# Autodesk Inventor assembly: SCHUNK- 1321170 Co-act EGP-C 40-N-N-KTOE, 0
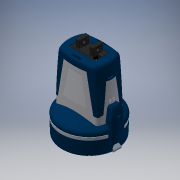
[picture p0: Inventor's stored thumbnail of the model, 180x180]
Saved by Autodesk Inventor 2019 (Build 230136000, 136)
## iProperties
Category: PARTsolutions
Company: SCHUNK
Created: 2022-08-29
Part Number: SCHUNK- 1321170 Co-act EGP-C 40-N-N-KTOE, 0
Catalog Web Link: www.cadenas.de
Description: Co-act EGP-C-Collaborating gripper for small components
Vendor: SCHUNK
Document SubType Name: Assembly
Designer: psAdmin
Manufacturer: SCHUNK
Mass: 620 g
Surface Area: 1018.14 cm^2
Volume: 436.323 cm^3
Density: 1.42097 g/cm^3
Title: SCHUNK-1321170 Co-act EGP-C 40-N-N-KTOE
Author: Cadenas PARTsolutions
Comments: Collaborating gripper for small components
PSOL_IDENT_0: {$CADENAS_DATA/23d-libs/schunk/greifsysteme/greifmodule/co_act/co_act_egp_c/co_act_egp_c_asm_at.prj}
PSOL_IDENT_1: ,248 {VTYP=3D},{STYP=ASSTAB},{NB=SCHUNK- 1321170 Co-act EGP-C 40-N-N-KTOE, 0},{LINA=SCHUNK-1321170 C
PSOL_IDENT_2: o-act EGP-C 40-N-N-KTOE},{NN=Co-act EGP-C},{DATE=01.06.2022 15:24:31},{GEOMDATE=27.04.2022 08:42:34}
PSOL_IDENT_3: ,{VERSION=},{LINEID=20},{WBVAR=HUB},{WBNUMERIC=HUB}  {NB=SCHUNK- 1321170 Co-act EGP-C 40-N-N-KTOE, 0
PSOL_IDENT_4: },{LINA=SCHUNK-1321170 Co-act EGP-C 40-N-N-KTOE},{KT=DUMMY},{IDNR=1321170},{TYP=Co-act EGP-C 40-N-N-
PSOL_IDENT_5: KTOE},{ONLINE=Zur Produktseite},{INFOXX=https://schunk.com/gb_en/gripping-systems/product/63294-0},{
PSOL_IDENT_6: HUB=0},{CALC=../../../../produktbilder/icons/im0023672.png},{EPLAN=../../../../produktbilder/icons/i
PSOL_IDENT_7: m0021678.png},{HUBMAX=6.000},{PARTSERVER=1.000},{TYPBG=2.000},{TYP1=1.000},{TYPFLA=2.000},{WFLA=30.0
PSOL_IDENT_8: 00},{TYPEGP=EGP 40-N-N-B},{ROBOTER=KUKA LBR iiwa 7/14},{FLANSCH=Medien-Flansch Touch elektrisch},{LE
PSOL_IDENT_9: D=integriert},{FARBEN=Grün, Gelb, Rot},{SENSOREN=Ja, 2-fach induktiv},{HUBBACKE=6},{GREIFKRAFT=35/14
PSOL_IDENT_10: 0},{KRAFTPROBACKE=17.5/70},{WKSTGEWICHT=0.700},{FINGERLAENGE=50},{MASSEFINGER=0.080},{WIEDERHOLGENAU
PSOL_IDENT_11: I=0.020},{SCHLIESSOEFFNUN=0.2/0.2},{EIGENMASSE=0.620},{UMGEBUNGSTEMPER=5/55},{SCHUTZART=30},{KABELST
PSOL_IDENT_12: ECKEREND=M12},{KABELLAENGE=70},{NENNSPANN=24},{NENNSTROM=0.200},{MAXSTROM=2.000},{REGLERELEKTRONI=in
PSOL_IDENT_13: tegriert},{KOMMUNIKATIONSS=Digitale I/O},{ANZDIGITALEIO=4/2},{HOEHE=118.000},{HEGP=88.500},{CALCXX=h
PSOL_IDENT_14: ttps://schunk.com/de_de/services/digitale-services/berechnungs-und-auslegungstool-greifen/},{CALCXXX=
PSOL_IDENT_15: https://schunk.com/de_de/services/digitale-services/berechnungs-und-auslegungstool-greifen/},{EPLANX
PSOL_IDENT_16: X=https://eplandata.de/portal/portal.php?action=part-viewc&edpp=1.0&ev=1.9.11&lang=de_DE&clang=de_DE
PSOL_IDENT_17: &mf=SNK&lastmpg=.&mcat=_eplan&tab=c&mcatsel=SNK},{EPLANXXX=https://eplandata.de/portal/portal.php?ac
PSOL_IDENT_18: tion=part-viewc&edpp=1.0&ev=1.9.11&lang=de_DE&clang=de_DE&mf=SNK&lastmpg=.&mcat=_eplan&tab=c&mcatsel=
PSOL_IDENT_19: SNK},{CNSCTN=84798997},{EDZ=snk.1321170},{EPIMID=63294},{PPATH=co_act_egp_c_asmsbl.prj}
NB: SCHUNK- 1321170 Co-act EGP-C 40-N-N-KTOE, 0
NN: Co-act EGP-C
NT: Collaborating gripper for small components
NBSYN: SCHUNK- $IDNR. $TYP., $HUB.
LINA: SCHUNK-1321170 Co-act EGP-C 40-N-N-KTOE
CATALOG: SCHUNK
IDNR: 1321170
TYP: Co-act EGP-C 40-N-N-KTOE
ONLINE: To the product page
HUB: 0
CALC: ../../../../produktbilder/icons/im0023672.png
EPLAN: ../../../../produktbilder/icons/im0021678.png
ROBOTER: KUKA LBR iiwa 7/14
FLANSCH: Media flange touch electric
LED: integrated
FARBEN: green, yellow, red
SENSOREN: yes, inductive in two directions
HUBBACKE: 6
GREIFKRAFT: 35/140
KRAFTPROBACKE: 17.5/70
WKSTGEWICHT: 0.7
FINGERLAENGE: 50
MASSEFINGER: 0.08
WIEDERHOLGENAUI: 0.02
SCHLIESSOEFFNUN: 0.2/0.2
EIGENMASSE: 0.62
UMGEBUNGSTEMPER: 5/55
SCHUTZART: 30
KABELSTECKEREND: M12
KABELLAENGE: 70
NENNSPANN: 24
NENNSTROM: 0.2
MAXSTROM: 2
REGLERELEKTRONI: integrated
KOMMUNIKATIONSS: digital I/O
ANZDIGITALEIO: 4/2
CNSCTN: 84798997
SUPPLIER: SCHUNK
ARTICLENO: SCHUNK- 1321170 Co-act EGP-C 40-N-N-KTOE, 0
BOMINFO: SCHUNK-1321170 Co-act EGP-C 40-N-N-KTOE
CREATOR: CADENAS GmbH
## Documents named in this file (11)
- e:\temp\worker_COMMON_2\temp\exporttempdir_6540_146_MRx3B\format_0\SCHUNK- 1321170 Co-act EGP-C 40-N-N-KTOE, 0.iam
- e:\temp\worker_COMMON_2\temp\exporttempdir_6540_146_MRx3B\format_0\Co-act EGP-C 40 Modell 1.ipt
- e:\temp\worker_COMMON_2\temp\exporttempdir_6540_146_MRx3B\format_0\SCHUNK-1013180-ISO-1-50-M6 Universalflansch Co-act-EGP-C.ipt
- e:\temp\worker_COMMON_2\temp\exporttempdir_6540_146_MRx3B\format_0\SCHUNK-9905502 Typenschild 9x24x0_3.ipt
- e:\temp\worker_COMMON_2\temp\exporttempdir_6540_146_MRx3B\format_0\SCHUNK-5521120 Gehaeuse EGP 40.ipt
- e:\temp\worker_COMMON_2\temp\exporttempdir_6540_146_MRx3B\format_0\SCHUNK-SNT016581 Stecker EGP.ipt
- e:\temp\worker_COMMON_2\temp\exporttempdir_6540_146_MRx3B\format_0\SCHUNK-9700901 Halter fuer NHS Du 4.ipt
- e:\temp\worker_COMMON_2\temp\exporttempdir_6540_146_MRx3B\format_0\SCHUNK-5521119 Finger EGP 40.ipt
- e:\temp\worker_COMMON_2\temp\exporttempdir_6540_146_MRx3B\format_0\SCHUNK-9962713 Bracket MPG 40.ipt
- e:\temp\worker_COMMON_2\temp\exporttempdir_6540_146_MRx3B\format_0\SCHUNK-9965221-Scheibe D4_5.ipt
- e:\temp\worker_COMMON_2\temp\exporttempdir_6540_146_MRx3B\format_0\SCHUNK-5509536 Huelse MPG 40.ipt
## Components (18 placed, 10 different names)
1. Co-act EGP-C 40 Modell 1:1 — fla_XY@1 <-> fla_XY@2, fla_Z@1 <-> fla_Z@2, fla_YZ@1 <-> fla_YZ@2, typ_XY@1 <-> aluschild_XY@3, typ_Z@1 <-> aluschild_Z@3, typ_YZ@1 <-> aluschild_YZ@3
2. SCHUNK-1013180-ISO-1-50-M6 Universalflansch Co-act-EGP-C:1 — fla_XY@1 <-> fla_XY@2, fla_Z@1 <-> fla_Z@2, fla_YZ@1 <-> fla_YZ@2
3. SCHUNK-9905502 Typenschild 9x24x0_3:1 — typ_XY@1 <-> aluschild_XY@3, typ_Z@1 <-> aluschild_Z@3, typ_YZ@1 <-> aluschild_YZ@3
4. SCHUNK-5521120 Gehaeuse EGP 40:1 — hal_nhs_1_XY@4 <-> as_nhs_02_XY@6, hal_nhs_1_Z@4 <-> as_nhs_02_Z@6, hal_nhs_1_YZ@4 <-> as_nhs_02_YZ@6, fin_1_XY@4 <-> HUB_XY@8, fin_1_Z@4 <-> HUB_Z@8, fin_1_YZ@4 <-> HUB_YZ@8, fin_2_XY@4 <-> HUB_XY@13, fin_2_Z@4 <-> HUB_Z@13, fin_2_YZ@4 <-> HUB_YZ@13, typ_XY@4 <-> aluschild_XY@18, typ_Z@4 <-> aluschild_Z@18, typ_YZ@4 <-> aluschild_YZ@18
5. SCHUNK-SNT016581 Stecker EGP:1
6. SCHUNK-9700901 Halter fuer NHS Du 4:1 — hal_nhs_1_XY@4 <-> as_nhs_02_XY@6, hal_nhs_1_Z@4 <-> as_nhs_02_Z@6, hal_nhs_1_YZ@4 <-> as_nhs_02_YZ@6
7. SCHUNK-9700901 Halter fuer NHS Du 4:2
8. SCHUNK-5521119 Finger EGP 40:1 — fin_1_XY@4 <-> HUB_XY@8, fin_1_Z@4 <-> HUB_Z@8, fin_1_YZ@4 <-> HUB_YZ@8, hal_1_XY@8 <-> hal_XY@9, hal_1_Z@8 <-> hal_Z@9, hal_1_YZ@8 <-> hal_YZ@9, hal_2_XY@8 <-> hal_XY@11, hal_2_Z@8 <-> hal_Z@11, hal_2_YZ@8 <-> hal_YZ@11
9. SCHUNK-9962713 Bracket MPG 40:1 — hal_1_XY@8 <-> hal_XY@9, hal_1_Z@8 <-> hal_Z@9, hal_1_YZ@8 <-> hal_YZ@9, s01_XY@9 <-> hal_XY@10, s01_Z@9 <-> hal_Z@10, s01_YZ@9 <-> hal_YZ@10
10. SCHUNK-9965221-Scheibe D4_5:1 — s01_XY@9 <-> hal_XY@10, s01_Z@9 <-> hal_Z@10, s01_YZ@9 <-> hal_YZ@10
11. SCHUNK-9962713 Bracket MPG 40:2 — hal_2_XY@8 <-> hal_XY@11, hal_2_Z@8 <-> hal_Z@11, hal_2_YZ@8 <-> hal_YZ@11, s01_XY@11 <-> hal_XY@12, s01_Z@11 <-> hal_Z@12, s01_YZ@11 <-> hal_YZ@12
12. SCHUNK-9965221-Scheibe D4_5:2 — s01_XY@11 <-> hal_XY@12, s01_Z@11 <-> hal_Z@12, s01_YZ@11 <-> hal_YZ@12
13. SCHUNK-5521119 Finger EGP 40:2 — fin_2_XY@4 <-> HUB_XY@13, fin_2_Z@4 <-> HUB_Z@13, fin_2_YZ@4 <-> HUB_YZ@13, hal_1_XY@13 <-> hal_XY@14, hal_1_Z@13 <-> hal_Z@14, hal_1_YZ@13 <-> hal_YZ@14, hal_2_XY@13 <-> hal_XY@16, hal_2_Z@13 <-> hal_Z@16, hal_2_YZ@13 <-> hal_YZ@16
14. SCHUNK-9962713 Bracket MPG 40:3 — hal_1_XY@13 <-> hal_XY@14, hal_1_Z@13 <-> hal_Z@14, hal_1_YZ@13 <-> hal_YZ@14, s01_XY@14 <-> hal_XY@15, s01_Z@14 <-> hal_Z@15, s01_YZ@14 <-> hal_YZ@15
15. SCHUNK-9965221-Scheibe D4_5:3 — s01_XY@14 <-> hal_XY@15, s01_Z@14 <-> hal_Z@15, s01_YZ@14 <-> hal_YZ@15
16. SCHUNK-9962713 Bracket MPG 40:4 — hal_2_XY@13 <-> hal_XY@16, hal_2_Z@13 <-> hal_Z@16, hal_2_YZ@13 <-> hal_YZ@16, s01_XY@16 <-> hul_XY@17, s01_Z@16 <-> hul_Z@17, s01_YZ@16 <-> hul_YZ@17
17. SCHUNK-5509536 Huelse MPG 40:1 — s01_XY@16 <-> hul_XY@17, s01_Z@16 <-> hul_Z@17, s01_YZ@16 <-> hul_YZ@17
18. SCHUNK-9905502 Typenschild 9x24x0_3:2 — typ_XY@4 <-> aluschild_XY@18, typ_Z@4 <-> aluschild_Z@18, typ_YZ@4 <-> aluschild_YZ@18
## Relationships (42: Mate 18, Angle 14, Flush 10)
- fla_XY@1 <-> fla_XY@2 [Flush]: Co-act EGP-C 40 Modell 1:1 ↔ SCHUNK-1013180-ISO-1-50-M6 Universalflansch Co-act-EGP-C:1
- fla_Z@1 <-> fla_Z@2 [Mate]: Co-act EGP-C 40 Modell 1:1 ↔ SCHUNK-1013180-ISO-1-50-M6 Universalflansch Co-act-EGP-C:1
- fla_YZ@1 <-> fla_YZ@2 [Angle] (-30 deg): Co-act EGP-C 40 Modell 1:1 ↔ SCHUNK-1013180-ISO-1-50-M6 Universalflansch Co-act-EGP-C:1
- typ_XY@1 <-> aluschild_XY@3 [Flush] (0.6 mm): Co-act EGP-C 40 Modell 1:1 ↔ SCHUNK-9905502 Typenschild 9x24x0_3:1
- typ_Z@1 <-> aluschild_Z@3 [Mate]: Co-act EGP-C 40 Modell 1:1 ↔ SCHUNK-9905502 Typenschild 9x24x0_3:1
- typ_YZ@1 <-> aluschild_YZ@3 [Angle] (0 deg): Co-act EGP-C 40 Modell 1:1 ↔ SCHUNK-9905502 Typenschild 9x24x0_3:1
- hal_nhs_1_XY@4 <-> as_nhs_02_XY@6 [Flush]: SCHUNK-5521120 Gehaeuse EGP 40:1 ↔ SCHUNK-9700901 Halter fuer NHS Du 4:1
- hal_nhs_1_Z@4 <-> as_nhs_02_Z@6 [Mate]: SCHUNK-5521120 Gehaeuse EGP 40:1 ↔ SCHUNK-9700901 Halter fuer NHS Du 4:1
- hal_nhs_1_YZ@4 <-> as_nhs_02_YZ@6 [Angle] (0 deg): SCHUNK-5521120 Gehaeuse EGP 40:1 ↔ SCHUNK-9700901 Halter fuer NHS Du 4:1
- fin_1_XY@4 <-> HUB_XY@8 [Flush]: SCHUNK-5521120 Gehaeuse EGP 40:1 ↔ SCHUNK-5521119 Finger EGP 40:1
- fin_1_Z@4 <-> HUB_Z@8 [Mate]: SCHUNK-5521120 Gehaeuse EGP 40:1 ↔ SCHUNK-5521119 Finger EGP 40:1
- fin_1_YZ@4 <-> HUB_YZ@8 [Angle] (0 deg): SCHUNK-5521120 Gehaeuse EGP 40:1 ↔ SCHUNK-5521119 Finger EGP 40:1
- hal_1_XY@8 <-> hal_XY@9 [Flush]: SCHUNK-5521119 Finger EGP 40:1 ↔ SCHUNK-9962713 Bracket MPG 40:1
- hal_1_Z@8 <-> hal_Z@9 [Mate]: SCHUNK-5521119 Finger EGP 40:1 ↔ SCHUNK-9962713 Bracket MPG 40:1
- hal_1_YZ@8 <-> hal_YZ@9 [Angle] (0 deg): SCHUNK-5521119 Finger EGP 40:1 ↔ SCHUNK-9962713 Bracket MPG 40:1
- s01_XY@9 <-> hal_XY@10 [Flush]: SCHUNK-9962713 Bracket MPG 40:1 ↔ SCHUNK-9965221-Scheibe D4_5:1
- s01_Z@9 <-> hal_Z@10 [Mate]: SCHUNK-9962713 Bracket MPG 40:1 ↔ SCHUNK-9965221-Scheibe D4_5:1
- s01_YZ@9 <-> hal_YZ@10 [Angle] (0 deg): SCHUNK-9962713 Bracket MPG 40:1 ↔ SCHUNK-9965221-Scheibe D4_5:1
- hal_2_XY@8 <-> hal_XY@11 [Mate]: SCHUNK-5521119 Finger EGP 40:1 ↔ SCHUNK-9962713 Bracket MPG 40:2
- hal_2_Z@8 <-> hal_Z@11 [Mate]: SCHUNK-5521119 Finger EGP 40:1 ↔ SCHUNK-9962713 Bracket MPG 40:2
- hal_2_YZ@8 <-> hal_YZ@11 [Angle] (0 deg): SCHUNK-5521119 Finger EGP 40:1 ↔ SCHUNK-9962713 Bracket MPG 40:2
- s01_XY@11 <-> hal_XY@12 [Flush]: SCHUNK-9962713 Bracket MPG 40:2 ↔ SCHUNK-9965221-Scheibe D4_5:2
- s01_Z@11 <-> hal_Z@12 [Mate]: SCHUNK-9962713 Bracket MPG 40:2 ↔ SCHUNK-9965221-Scheibe D4_5:2
- s01_YZ@11 <-> hal_YZ@12 [Angle] (0 deg): SCHUNK-9962713 Bracket MPG 40:2 ↔ SCHUNK-9965221-Scheibe D4_5:2
- fin_2_XY@4 <-> HUB_XY@13 [Mate]: SCHUNK-5521120 Gehaeuse EGP 40:1 ↔ SCHUNK-5521119 Finger EGP 40:2
- fin_2_Z@4 <-> HUB_Z@13 [Mate]: SCHUNK-5521120 Gehaeuse EGP 40:1 ↔ SCHUNK-5521119 Finger EGP 40:2
- fin_2_YZ@4 <-> HUB_YZ@13 [Angle] (180 deg): SCHUNK-5521120 Gehaeuse EGP 40:1 ↔ SCHUNK-5521119 Finger EGP 40:2
- hal_1_XY@13 <-> hal_XY@14 [Flush]: SCHUNK-5521119 Finger EGP 40:2 ↔ SCHUNK-9962713 Bracket MPG 40:3
- hal_1_Z@13 <-> hal_Z@14 [Mate]: SCHUNK-5521119 Finger EGP 40:2 ↔ SCHUNK-9962713 Bracket MPG 40:3
- hal_1_YZ@13 <-> hal_YZ@14 [Angle] (0 deg): SCHUNK-5521119 Finger EGP 40:2 ↔ SCHUNK-9962713 Bracket MPG 40:3
- s01_XY@14 <-> hal_XY@15 [Flush]: SCHUNK-9962713 Bracket MPG 40:3 ↔ SCHUNK-9965221-Scheibe D4_5:3
- s01_Z@14 <-> hal_Z@15 [Mate]: SCHUNK-9962713 Bracket MPG 40:3 ↔ SCHUNK-9965221-Scheibe D4_5:3
- s01_YZ@14 <-> hal_YZ@15 [Angle] (0 deg): SCHUNK-9962713 Bracket MPG 40:3 ↔ SCHUNK-9965221-Scheibe D4_5:3
- hal_2_XY@13 <-> hal_XY@16 [Mate]: SCHUNK-5521119 Finger EGP 40:2 ↔ SCHUNK-9962713 Bracket MPG 40:4
- hal_2_Z@13 <-> hal_Z@16 [Mate]: SCHUNK-5521119 Finger EGP 40:2 ↔ SCHUNK-9962713 Bracket MPG 40:4
- hal_2_YZ@13 <-> hal_YZ@16 [Angle] (0 deg): SCHUNK-5521119 Finger EGP 40:2 ↔ SCHUNK-9962713 Bracket MPG 40:4
- s01_XY@16 <-> hul_XY@17 [Flush]: SCHUNK-9962713 Bracket MPG 40:4 ↔ SCHUNK-5509536 Huelse MPG 40:1
- s01_Z@16 <-> hul_Z@17 [Mate]: SCHUNK-9962713 Bracket MPG 40:4 ↔ SCHUNK-5509536 Huelse MPG 40:1
- s01_YZ@16 <-> hul_YZ@17 [Angle] (0 deg): SCHUNK-9962713 Bracket MPG 40:4 ↔ SCHUNK-5509536 Huelse MPG 40:1
- typ_XY@4 <-> aluschild_XY@18 [Mate]: SCHUNK-5521120 Gehaeuse EGP 40:1 ↔ SCHUNK-9905502 Typenschild 9x24x0_3:2
- typ_Z@4 <-> aluschild_Z@18 [Mate]: SCHUNK-5521120 Gehaeuse EGP 40:1 ↔ SCHUNK-9905502 Typenschild 9x24x0_3:2
- typ_YZ@4 <-> aluschild_YZ@18 [Angle] (0 deg): SCHUNK-5521120 Gehaeuse EGP 40:1 ↔ SCHUNK-9905502 Typenschild 9x24x0_3:2
